# Autodesk Inventor assembly: Main
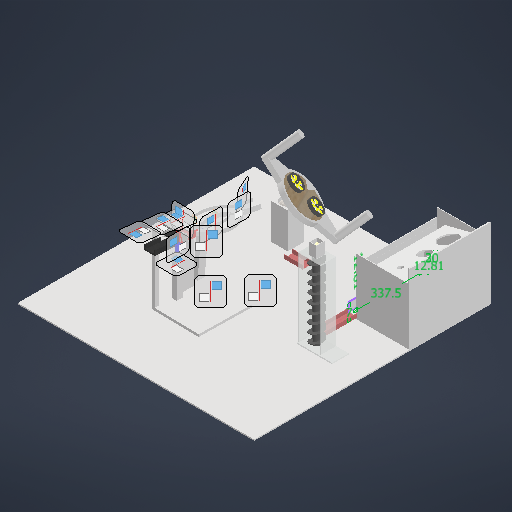
[picture p0: Inventor's stored thumbnail of the model, 512x512]
Saved by Autodesk Inventor 2026.2 (Build 302298000, 298)
## iProperties
Created: 2026-03-06
Part Number: Main
Document SubType Name: Assembly
Designer: danda
Author: danda
## Documents named in this file (8)
- C:\Users\danda\BOM-project\Project\CAD\Main.iam
- C:\Users\danda\BOM-project\Project\CAD\baseb.ipt
- C:\Users\danda\BOM-project\Project\CAD\sorting\Assembly2.iam
- C:\Users\danda\BOM-project\Project\CAD\Shooting Mechanism CAD\Shooting Mechanism Assembly.iam
- C:\Users\danda\BOM-project\Project\CAD\collectingbox.ipt
- C:\Users\danda\BOM-project\Project\CAD\5mmhieght.ipt
- C:\Users\danda\BOM-project\Project\CAD\collectingslide.ipt
- C:\Users\danda\BOM-project\Project\CAD\Lifting\Lifting\liftingAssembly2.iam
## Components (7 placed, 7 different names)
1. baseb:1 — Mate:1, Mate:2, Mate:3, Flush:1, Mate:6, Mate:9, Mate:11, Mate:14, Flush:5, Flush:6, Mate:15
2. Shooting Mechanism Assembly:1 [sub-assembly] — Mate:14, Flush:6
3. Assembly2:3 [sub-assembly] — Mate:6
4. collectingbox:1 — Flush:1, Mate:10, Flush:2, Flush:3, Flush:5, Flush:7
5. 5mmhieght:1 — Mate:9, Mate:10, Flush:2, Flush:3, Mate:12
6. collectingslide:1 — Mate:11, Mate:12, Mate:16, Flush:7, Flush:8
7. liftingAssembly2:1 [sub-assembly] — Mate:15, Mate:16, Flush:8
## Relationships (18: Mate 11, Flush 7)
- Mate:1: baseb:1
- Mate:2: baseb:1
- Mate:3: baseb:1
- Flush:1: baseb:1 ↔ collectingbox:1
- Mate:6: baseb:1 ↔ Assembly2:3
- Mate:9: baseb:1 ↔ 5mmhieght:1
- Mate:10: collectingbox:1 ↔ 5mmhieght:1
- Flush:2: collectingbox:1 ↔ 5mmhieght:1
- Flush:3: collectingbox:1 ↔ 5mmhieght:1
- Mate:11: baseb:1 ↔ collectingslide:1
- Mate:12: 5mmhieght:1 ↔ collectingslide:1
- Mate:14: baseb:1 ↔ Shooting Mechanism Assembly:1
- Flush:5: baseb:1 ↔ collectingbox:1
- Flush:6 (170 mm): baseb:1 ↔ Shooting Mechanism Assembly:1
- Mate:15: baseb:1 ↔ liftingAssembly2:1
- Mate:16: collectingslide:1 ↔ liftingAssembly2:1
- Flush:7: collectingbox:1 ↔ collectingslide:1
- Flush:8: collectingslide:1 ↔ liftingAssembly2:1
